# Autodesk Inventor assembly: gripper
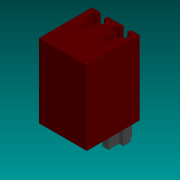
[picture p0: Inventor's stored thumbnail of the model, 180x180]
Saved by Autodesk Inventor 2020.3 (Build 243373000, 373)
## iProperties
Created: 2020-05-25
Part Number: gripper
Document SubType Name: Assembly
Designer: Svend
Author: Svend
## Documents named in this file (3)
- C:\Users\Svend\OneDrive\Documents\GitHub\BeerMinder\3D-model\gripper\gripper.iam
- C:\Users\Svend\OneDrive\Documents\GitHub\BeerMinder\3D-model\gripper\slider.ipt
- C:\Users\Svend\OneDrive\Documents\GitHub\BeerMinder\3D-model\gripper\grippershape.ipt
## Components (3 placed, 2 different names)
1. slider:1 — Angle:1, Flush:1, Mate:1
2. slider:2 — Angle:1, Flush:1, Mate:1, Mate:2, Mate:3
3. grippershape:1 — Mate:2, Mate:3
## Relationships (5: Mate 3, Angle 1, Flush 1)
- Angle:1 (0 deg): slider:1 ↔ slider:2
- Flush:1: slider:1 ↔ slider:2
- Mate:1 (15.45 mm): slider:1 ↔ slider:2
- Mate:2 (0.1 mm): slider:2 ↔ grippershape:1
- Mate:3 (0.1 mm): slider:2 ↔ grippershape:1
